# Autodesk Inventor assembly: bottom_cover
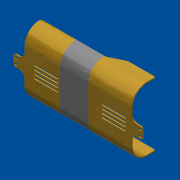
[picture p0: Inventor's stored thumbnail of the model, 180x180]
Saved by Autodesk Inventor 2019 (Build 230136000, 136)
## iProperties
Created: 2020-10-07
Part Number: bottom_cover
Document SubType Name: Assembly
Designer: ewdia
Author: ewdia
## Documents named in this file (4)
- C:\Users\ewdia\Downloads\balam_assembly parts\bottom_cover\bottom_cover.iam
- C:\Users\ewdia\Downloads\balam_assembly parts\bottom_cover\Imported Components\BottomCover_1\BottomCover_1.ipt
- C:\Users\ewdia\Downloads\balam_assembly parts\bottom_cover\Imported Components\BottomCover_2\BottomCover_2.ipt
- C:\Users\ewdia\Downloads\balam_assembly parts\bottom_cover\Imported Components\BottomCoverSpacer\BottomCoverSpacer.ipt
## Components (3 placed, 3 different names)
1. BottomCover_1:1 — Rigid:1
2. BottomCover_2:1 — Rigid:2
3. BottomCoverSpacer:1 — Rigid:1, Rigid:2
## Relationships (2: WeldJoint 2)
- Rigid:1 [WeldJoint]: BottomCover_1:1 ↔ BottomCoverSpacer:1
- Rigid:2 [WeldJoint]: BottomCover_2:1 ↔ BottomCoverSpacer:1
